# Autodesk Inventor assembly: PSCSPJ6-6
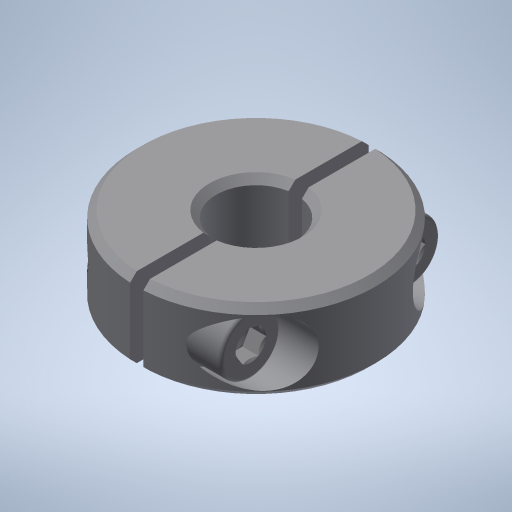
[picture p0: Inventor's stored thumbnail of the model, 512x512]
Saved by Autodesk Inventor 2024.1 (Build 281209000, 209)
## iProperties
Created: 2023-10-07
Part Number: PSCSPJ6-6
Catalog Web Link: www.cadenas.de
Description: SCSPJ, PSCSPJ, SSCSPJ, SCNPAJ, SCNPAWJ-Set Collars - Separate - Standard Compact Type
Vendor: MISUMI
Document SubType Name: Assembly
Designer: psAdmin
Manufacturer: MISUMI
Mass: 1.19599 g
Surface Area: 13.6586 cm^2
Volume: 1.19599 cm^3
Density: 1 g/cm^3
Category: PARTsolutions
Company: MISUMI
PSOL_IDENT_0: {$CADENAS_DATA/23d-libs/misumi/metric/03_set_collars/scspj_asmtab.prj},211 {VTYP=3D},{STYP=ASSTAB},{
PSOL_IDENT_1: NB=PSCSPJ6-6},{LINA=PSCSPJ6-6},{NN=SCSPJ, PSCSPJ, SSCSPJ, SCNPAJ, SCNPAWJ},{DATE=18.06.2021 05:39:41
PSOL_IDENT_2: },{GEOMDATE=08.06.2021 05:32:32},{VERSION=},{LINEID=300},{WBVAR=MAT,ST},{WBNUMERIC=}  {NB=PSCSPJ6-6}
PSOL_IDENT_3: ,{LINA=PSCSPJ6-6},{KT=DUMMY},{PN=PSCSPJ6-6},{TYPE=PSCSPJ},{MAT=1},{MATALG='1','1045 Carbon Steel','2'
PSOL_IDENT_4: ,'SUS304 Equivalent','3','2017 Aluminum Alloy'},{ST=2},{AC=Hexagon Socket Head Cap Screw 2 Pc. (SUS)
PSOL_IDENT_5: },{D=6},{B=6},{D1=18},{M=M2.6},{M1=2.6},{STALG='1','Black Oxide','2','Electroless Nickel Plating'},{
PSOL_IDENT_6: DD=2.9},{R=2.45},{W=1.0},{X=6.0},{Y=3},{C=0.5},{L=6},{LS=6},{PPATH=scspj/scspj_templ.prj}
NB: PSCSPJ6-6
NN: SCSPJ, PSCSPJ, SSCSPJ, SCNPAJ, SCNPAWJ
NT: Set Collars - Separate - Standard Compact Type
NBSYN: $PN.
LINA: PSCSPJ6-6
CATALOG: Misumi
PN: PSCSPJ6-6
MAT: 1045 Carbon Steel
ST: Electroless Nickel Plating
AC: Hexagon Socket Head Cap Screw 2 Pc. (SUS)
D: 6
B: 6
D1: 18
M: M2.6
DD: 2.9
R: 2.45
W: 1
X: 6
Y: 3
SUPPLIER: MISUMI
ARTICLENO: PSCSPJ6-6
BOMINFO: PSCSPJ6-6
CREATOR: CADENAS GmbH
Title: PSCSPJ6-6
Author: Cadenas PARTsolutions
Comments: Set Collars - Separate - Standard Compact Type
## Documents named in this file (4)
- C:\Users\haruy\OneDrive - Kyushu University\cad\000_parts\セットカラー\setcolor-6-18\PSCSPJ6-6.iam
- C:\Users\haruy\OneDrive - Kyushu University\cad\000_parts\セットカラー\setcolor-6-18\PSCSPJ6-6b.ipt
- C:\Users\haruy\OneDrive - Kyushu University\cad\000_parts\セットカラー\setcolor-6-18\M2_6x66.ipt
- C:\Users\haruy\OneDrive - Kyushu University\cad\000_parts\セットカラー\setcolor-6-18\PSCSPJ6-6p.ipt
## Components (4 placed, 3 different names)
1. PSCSPJ6-6b:1 — body_screw_Z@1 <-> IP4_Z@2, body_screw2_Z@1 <-> IP1_Z@3
2. M2_6x66:1 — body_screw_Z@1 <-> IP4_Z@2
3. M2_6x66:2 — body_screw2_Z@1 <-> IP1_Z@3
4. PSCSPJ6-6p:1
## Relationships (2: Mate 2)
- body_screw_Z@1 <-> IP4_Z@2 [Mate]: PSCSPJ6-6b:1 ↔ M2_6x66:1
- body_screw2_Z@1 <-> IP1_Z@3 [Mate]: PSCSPJ6-6b:1 ↔ M2_6x66:2
